# Autodesk Inventor assembly: uMule-Koło
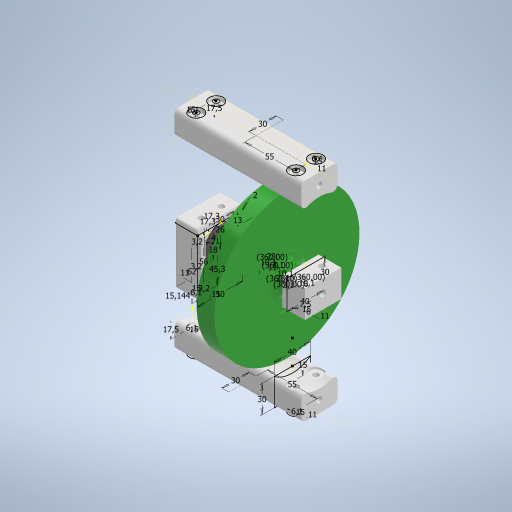
[picture p0: Inventor's stored thumbnail of the model, 512x512]
Saved by Autodesk Inventor 2024.3 (Build 283343000, 343)
## iProperties
Created: 2024-10-21
Part Number: uMule-Koło
Document SubType Name: Assembly
Designer: owozn
Author: owozn
## Documents named in this file (6)
- C:\Users\owozn\Documents\Nauka\Studia\mgr\Semestr_3\Magisterka\temp\uMule\mechanics\subsets\wheel\uMule-wheel_complete.iam
- C:\Users\owozn\Documents\Nauka\Studia\mgr\Semestr_3\Magisterka\temp\uMule\mechanics\subsets\wheel\uMule-wheel.ipt
- C:\Users\owozn\Documents\Nauka\Studia\mgr\Semestr_3\Magisterka\temp\uMule\mechanics\subsets\wheel\rx64H.ipt
- C:\Users\owozn\Documents\Nauka\Studia\mgr\Semestr_3\Magisterka\temp\uMule\mechanics\subsets\wheel\uMule-wheel_support.ipt
- C:\Users\owozn\Documents\Nauka\Studia\mgr\Semestr_3\Magisterka\temp\uMule\mechanics\subsets\wheel\uMule-wheel_limiter.ipt
- C:\Users\owozn\Documents\Nauka\Studia\mgr\Semestr_3\Magisterka\temp\uMule\mechanics\subsets\wheel\uMule-dx_top.ipt
## Components (7 placed, 5 different names)
1. uMule-wheel:1 — Mate:1, Mate:2, Mate:3, Mate:4, Mate:7
2. uMule-wheel:2 — Mate:1, Mate:2, Mate:3, Mate:5
3. rx64H:1 — Mate:4, Mate:5, Flush:2, Mate:15, Mate:16
4. uMule-wheel_support:1 — Mate:7, Mate:10, Flush:3, Flush:4
5. uMule-wheel_limiter:1 — Mate:10, Mate:11, Mate:12, Flush:4, Flush:6
6. uMule-wheel_limiter:2 — Mate:11, Mate:12, Flush:3, Flush:5, Flush:6
7. uMule-dx_top:1 — Flush:2, Mate:15, Mate:16, Flush:5
## Relationships (16: Mate 11, Flush 5)
- Mate:1: uMule-wheel:1 ↔ uMule-wheel:2
- Mate:2: uMule-wheel:1 ↔ uMule-wheel:2
- Mate:3: uMule-wheel:1 ↔ uMule-wheel:2
- Mate:4: uMule-wheel:1 ↔ rx64H:1
- Mate:5: uMule-wheel:2 ↔ rx64H:1
- Mate:7 (4 mm): uMule-wheel:1 ↔ uMule-wheel_support:1
- Mate:10: uMule-wheel_support:1 ↔ uMule-wheel_limiter:1
- Mate:11: uMule-wheel_limiter:1 ↔ uMule-wheel_limiter:2
- Mate:12: uMule-wheel_limiter:1 ↔ uMule-wheel_limiter:2
- Flush:2: rx64H:1 ↔ uMule-dx_top:1
- Mate:15: rx64H:1 ↔ uMule-dx_top:1
- Mate:16: rx64H:1 ↔ uMule-dx_top:1
- Flush:3 (100 mm): uMule-wheel_support:1 ↔ uMule-wheel_limiter:2
- Flush:4 (100 mm): uMule-wheel_support:1 ↔ uMule-wheel_limiter:1
- Flush:5 (5 mm): uMule-wheel_limiter:2 ↔ uMule-dx_top:1
- Flush:6: uMule-wheel_limiter:1 ↔ uMule-wheel_limiter:2
